# Autodesk Inventor assembly: MEMS I2S I
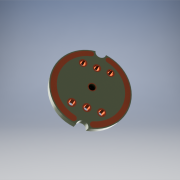
[picture p0: Inventor's stored thumbnail of the model, 180x180]
Saved by Autodesk Inventor 2016 SP2 (Build 200237200, 237)
## iProperties
Created: 2023-04-15
Part Number: MEMS I2S I
Document SubType Name: Assembly
Designer: Mark
Author: Mark
## Documents named in this file (5)
- G:\My Drive\NU2022\CAD - 3DPRT - SOFTWARE - MODELS\~SYNERGY PAC\UPC\ELECTRONIC PARTS - MODULES\MODULES\AUDIO\GRABCAD\MEMS I2S I.iam
- G:\My Drive\NU2022\CAD - 3DPRT - SOFTWARE - MODELS\~SYNERGY PAC\UPC\ELECTRONIC PARTS - MODULES\MODULES\AUDIO\INMP441 MEMS I2S MICROPHONE PCB.ipt
- G:\My Drive\NU2022\CAD - 3DPRT - SOFTWARE - MODELS\~SYNERGY PAC\UPC\ELECTRONIC PARTS - MODULES\MODULES\AUDIO\msm261s4030-mic-microphone-mems-digital-iis-i2s-1.snapshot.3\MSM261S4030.iam
- G:\My Drive\NU2022\CAD - 3DPRT - SOFTWARE - MODELS\~SYNERGY PAC\UPC\ELECTRONIC PARTS - MODULES\RESISTORS\ceramic-resistors-1.snapshot.1\Resistor 0402.ipt
- G:\My Drive\NU2022\CAD - 3DPRT - SOFTWARE - MODELS\~SYNERGY PAC\UPC\ELECTRONIC PARTS - MODULES\CAPACITORS\Ceramic Capacitors\C0402-T50-X7R.ipt
## Components (4 placed, 4 different names)
1. INMP441 MEMS I2S MICROPHONE PCB:1 — Mate:1, Mate:3, Mate:4, Mate:5
2. MSM261S4030:1 [sub-assembly] — Mate:1, Mate:3
3. Resistor 0402:1 — Mate:4
4. C0402-T50-X7R:1 — Mate:5
## Relationships (4: Mate 4)
- Mate:1: INMP441 MEMS I2S MICROPHONE PCB:1 ↔ MSM261S4030:1
- Mate:3: INMP441 MEMS I2S MICROPHONE PCB:1 ↔ MSM261S4030:1
- Mate:4: INMP441 MEMS I2S MICROPHONE PCB:1 ↔ Resistor 0402:1
- Mate:5: INMP441 MEMS I2S MICROPHONE PCB:1 ↔ C0402-T50-X7R:1
